# Autodesk Inventor assembly: KND-2610 Main way 01
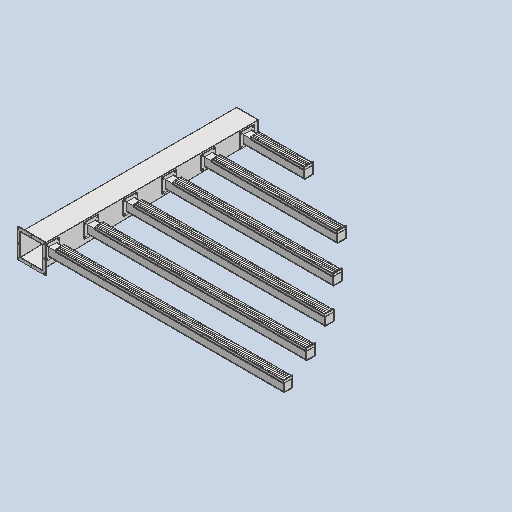
[picture p0: Inventor's stored thumbnail of the model, 512x512]
Saved by Autodesk Inventor 2026.2 (Build 302298000, 298)
## iProperties
Created: 2026-05-12
Part Number: KND-2610 Main way 01
Document SubType Name: Assembly
Designer: admin
Author: admin
## Documents named in this file (19)
- C:\Users\admin\Documents\Inventor\KND-DistribSystem\DRS_D1200\KND-2610 Main way 01.iam
- C:\Users\admin\Documents\Inventor\KND-DistribSystem\DRS_D1200\KND-1425 DrSysB Way FLANGE 01.ipt
- C:\Users\admin\Documents\Inventor\KND-DistribSystem\DRS_D1200\KND-1663 DrSysB way tube 4 01.ipt
- C:\Users\admin\Documents\Inventor\KND-DistribSystem\DRS_D1200\KND-1662 DrSysB way tube 2 01.ipt
- C:\Users\admin\Documents\Inventor\KND-DistribSystem\DRS_D1200\KND-1666 FDS 1000 CUP 1 01.ipt
- C:\Users\admin\Documents\Inventor\KND-DistribSystem\DRS_D1200\KND-1422 DrSysB diameter way up 01.ipt
- C:\Users\admin\Documents\Inventor\KND-DistribSystem\DRS_D1200\KND-1423 DrSysB diameter way down 01.ipt
- C:\Users\admin\Documents\Inventor\KND-DistribSystem\DRS_D1200\KND-1424 DrSysB diam way cup 01.ipt
- C:\Users\admin\Documents\Inventor\KND-DistribSystem\DRS_D1200\KND-1661 DrSysB way tube 1 01.ipt
- C:\Users\admin\Documents\Inventor\KND-DistribSystem\DRS_D1200\KND-5311 DrSysB roof 1 01.ipt
- C:\Users\admin\Documents\Inventor\KND-DistribSystem\DRS_D1200\KND-5321 DrSysB roof 2 01.ipt
- C:\Users\admin\Documents\Inventor\KND-DistribSystem\DRS_D1200\KND-5333 DrSysB roof 3 01.ipt
- C:\Users\admin\Documents\Inventor\KND-DistribSystem\DRS_D1200\KND-1664 DrSysB way tube 44 01.ipt
- C:\Users\admin\Documents\Inventor\KND-DistribSystem\DRS_D1200\KND-5335 DrSysB roof 33 01.ipt
- C:\Users\admin\Documents\Inventor\KND-DistribSystem\DRS_D1200\KND-1667 DrSysB way tube 5 01.ipt
- C:\Users\admin\Documents\Inventor\KND-DistribSystem\DRS_D1200\KND-5337 DrSysB roof 5 01.ipt
- C:\Users\admin\Documents\Inventor\KND-DistribSystem\DRS_D1200\KND-1668 DrSysB way tube 6 01.ipt
- C:\Users\admin\Documents\Inventor\KND-DistribSystem\DRS_D1200\KND-5338 DrSysB roof 6 01.ipt
- C:\Users\admin\Documents\Inventor\KND-DistribSystem\DRS_D1200\KND-1426 DrSysB Main way FLANGE 01.ipt
## Components (28 placed, 20 different names)
1. PRS 1425 DrSysB Way FLANGE_D1200:1 — Mate:34, Mate:40, Mate:41
2. PRS 1662 DrSysB way tube 4_D1200:1 — Mate:55, Mate:56, Mate:57, Mate:70, Flush:12, Mate:80, Mate:81, Flush:17, Mate:89, Flush:24
3. PRS 1662 DrSysB way tube 2_D1200:1 — Mate:52, Mate:53, Mate:54, Mate:67, Mate:68, Flush:11, Mate:78, Mate:79, Flush:16, Mate:88, Flush:22
4. PRS-1666 FDS 1000 CUP 1_D1200:1 — Rigid:17, Mate:15
5. PRS 1422 DrSysB diameter way up_D1200:1 — Flush:10, Flush:9, Mate:11, Rigid:23, Mate:94
6. PRS 1423 DrSysB diameter way down_D1200:1 — Rigid:23, Mate:16, Mate:17, Mate:18, Mate:34, Mate:52, Mate:53, Mate:54, Mate:55, Mate:56, Mate:57, Mate:58, Mate:59, Mate:60, Mate:61, Mate:62, Mate:63, Mate:64, Mate:65, Mate:66, Mate:69, Mate:71, Mate:73, Mate:75, Mate:77, Mate:93, Flush:31
7. PRS 1424 DrSysB diam way cup_D1200:1 — Flush:10, Flush:9, Mate:11
8. PRS 1425 DrSysB Way FLANGE_D1200:2 — Mate:69, Mate:78, Mate:79
9. PRS 1425 DrSysB Way FLANGE_D1200:3 — Mate:71, Mate:80, Mate:81
10. PRS 1661 DrSysB way tube 1_D1200:1 — Rigid:17, Mate:14, Flush:10, Mate:16, Mate:17, Mate:18, Mate:40, Mate:41
11. PRS 5311 DrSysB roof 1_D1200:1 — Mate:14, Flush:10, Mate:15
12. PRS 5321 DrSysB roof 2_D1200:1 — Mate:67, Mate:68, Flush:11, Flush:16, Flush:21
13. PRS 5333 DrSysB roof 3_D1200:1 — Mate:70, Flush:12, Flush:17, Flush:23
14. PRS 1662 DrSysB way tube 44_D1200:1 — Mate:58, Mate:59, Mate:60, Mate:72, Flush:13, Mate:82, Mate:83, Flush:18, Mate:90, Flush:26
15. PRS 5335 DrSysB roof 33_D1200:1 — Mate:72, Flush:13, Flush:18, Flush:25
16. PRS 1425 DrSysB Way FLANGE_D1200:7 — Mate:73, Mate:82, Mate:83
17. KND-1667 DrSysB way tube 5 01:1 — Mate:61, Mate:62, Mate:63, Mate:74, Flush:14, Mate:84, Mate:85, Flush:19, Mate:91, Flush:28
18. KND-5337 DrSysB roof 5 01:1 — Mate:74, Flush:14, Flush:19, Flush:27
19. KND-1425 DrSysB Way FLANGE 01:8 — Mate:75, Mate:84, Mate:85
20. KND-1668 DrSysB way tube 6 01:1 — Mate:64, Mate:65, Mate:66, Mate:76, Flush:15, Mate:86, Mate:87, Flush:20, Mate:92, Flush:30
21. KND-5338 DrSysB roof 6 01:1 — Mate:76, Flush:15, Flush:20, Flush:29
22. KND-1425 DrSysB Way FLANGE 01:9 — Mate:77, Mate:86, Mate:87
23. KND-1666 FDS 1000 CUP 1 01:2 — Mate:88, Flush:21, Flush:22
24. KND-1666 FDS 1000 CUP 1 01:3 — Mate:89, Flush:23, Flush:24
25. KND-1666 FDS 1000 CUP 1 01:4 — Mate:90, Flush:25, Flush:26
26. KND-1666 FDS 1000 CUP 1 01:5 — Mate:91, Flush:27, Flush:28
27. KND-1666 FDS 1000 CUP 1 01:6 — Mate:92, Flush:29, Flush:30
28. KND-1426 DrSysB Main way FLANGE 01:1 — Mate:93, Mate:94, Flush:31
## Relationships (78: Mate 52, Flush 24, WeldJoint 2)
- Flush:10 (1 mm): PRS 1422 DrSysB diameter way up_D1200:1 ↔ PRS 1424 DrSysB diam way cup_D1200:1
- Flush:9 (-1 mm): PRS 1422 DrSysB diameter way up_D1200:1 ↔ PRS 1424 DrSysB diam way cup_D1200:1
- Mate:11: PRS 1422 DrSysB diameter way up_D1200:1 ↔ PRS 1424 DrSysB diam way cup_D1200:1
- Rigid:23 [WeldJoint]: PRS 1422 DrSysB diameter way up_D1200:1 ↔ PRS 1423 DrSysB diameter way down_D1200:1
- Rigid:17 [WeldJoint]: PRS-1666 FDS 1000 CUP 1_D1200:1 ↔ PRS 1661 DrSysB way tube 1_D1200:1
- Mate:14 (10 mm): PRS 1661 DrSysB way tube 1_D1200:1 ↔ PRS 5311 DrSysB roof 1_D1200:1
- Flush:10: PRS 1661 DrSysB way tube 1_D1200:1 ↔ PRS 5311 DrSysB roof 1_D1200:1
- Mate:15: PRS-1666 FDS 1000 CUP 1_D1200:1 ↔ PRS 5311 DrSysB roof 1_D1200:1
- Mate:16: PRS 1423 DrSysB diameter way down_D1200:1 ↔ PRS 1661 DrSysB way tube 1_D1200:1
- Mate:17 (0.25 mm): PRS 1423 DrSysB diameter way down_D1200:1 ↔ PRS 1661 DrSysB way tube 1_D1200:1
- Mate:18 (0.25 mm): PRS 1423 DrSysB diameter way down_D1200:1 ↔ PRS 1661 DrSysB way tube 1_D1200:1
- Mate:34: PRS 1425 DrSysB Way FLANGE_D1200:1 ↔ PRS 1423 DrSysB diameter way down_D1200:1
- Mate:40 (0.1 mm): PRS 1425 DrSysB Way FLANGE_D1200:1 ↔ PRS 1661 DrSysB way tube 1_D1200:1
- Mate:41 (0.1 mm): PRS 1425 DrSysB Way FLANGE_D1200:1 ↔ PRS 1661 DrSysB way tube 1_D1200:1
- Mate:52: PRS 1662 DrSysB way tube 2_D1200:1 ↔ PRS 1423 DrSysB diameter way down_D1200:1
- Mate:53 (0.25 mm): PRS 1662 DrSysB way tube 2_D1200:1 ↔ PRS 1423 DrSysB diameter way down_D1200:1
- Mate:54 (0.25 mm): PRS 1662 DrSysB way tube 2_D1200:1 ↔ PRS 1423 DrSysB diameter way down_D1200:1
- Mate:55: PRS 1662 DrSysB way tube 4_D1200:1 ↔ PRS 1423 DrSysB diameter way down_D1200:1
- Mate:56 (0.25 mm): PRS 1662 DrSysB way tube 4_D1200:1 ↔ PRS 1423 DrSysB diameter way down_D1200:1
- Mate:57 (0.25 mm): PRS 1662 DrSysB way tube 4_D1200:1 ↔ PRS 1423 DrSysB diameter way down_D1200:1
- Mate:58: PRS 1423 DrSysB diameter way down_D1200:1 ↔ PRS 1662 DrSysB way tube 44_D1200:1
- Mate:59 (0.25 mm): PRS 1423 DrSysB diameter way down_D1200:1 ↔ PRS 1662 DrSysB way tube 44_D1200:1
- Mate:60 (0.25 mm): PRS 1423 DrSysB diameter way down_D1200:1 ↔ PRS 1662 DrSysB way tube 44_D1200:1
- Mate:61: PRS 1423 DrSysB diameter way down_D1200:1 ↔ KND-1667 DrSysB way tube 5 01:1
- Mate:62 (0.25 mm): PRS 1423 DrSysB diameter way down_D1200:1 ↔ KND-1667 DrSysB way tube 5 01:1
- Mate:63 (0.25 mm): PRS 1423 DrSysB diameter way down_D1200:1 ↔ KND-1667 DrSysB way tube 5 01:1
- Mate:64: PRS 1423 DrSysB diameter way down_D1200:1 ↔ KND-1668 DrSysB way tube 6 01:1
- Mate:65 (0.25 mm): PRS 1423 DrSysB diameter way down_D1200:1 ↔ KND-1668 DrSysB way tube 6 01:1
- Mate:66 (0.25 mm): PRS 1423 DrSysB diameter way down_D1200:1 ↔ KND-1668 DrSysB way tube 6 01:1
- Mate:67 (10 mm): PRS 1662 DrSysB way tube 2_D1200:1 ↔ PRS 5321 DrSysB roof 2_D1200:1
- Mate:68 (10 mm): PRS 1662 DrSysB way tube 2_D1200:1 ↔ PRS 5321 DrSysB roof 2_D1200:1
- Flush:11: PRS 1662 DrSysB way tube 2_D1200:1 ↔ PRS 5321 DrSysB roof 2_D1200:1
- Mate:69: PRS 1423 DrSysB diameter way down_D1200:1 ↔ PRS 1425 DrSysB Way FLANGE_D1200:2
- Mate:70 (10 mm): PRS 1662 DrSysB way tube 4_D1200:1 ↔ PRS 5333 DrSysB roof 3_D1200:1
- Flush:12: PRS 1662 DrSysB way tube 4_D1200:1 ↔ PRS 5333 DrSysB roof 3_D1200:1
- Mate:71: PRS 1423 DrSysB diameter way down_D1200:1 ↔ PRS 1425 DrSysB Way FLANGE_D1200:3
- Mate:72 (10 mm): PRS 1662 DrSysB way tube 44_D1200:1 ↔ PRS 5335 DrSysB roof 33_D1200:1
- Flush:13: PRS 1662 DrSysB way tube 44_D1200:1 ↔ PRS 5335 DrSysB roof 33_D1200:1
- Mate:73: PRS 1423 DrSysB diameter way down_D1200:1 ↔ PRS 1425 DrSysB Way FLANGE_D1200:7
- Mate:74 (10 mm): KND-1667 DrSysB way tube 5 01:1 ↔ KND-5337 DrSysB roof 5 01:1
- Flush:14: KND-1667 DrSysB way tube 5 01:1 ↔ KND-5337 DrSysB roof 5 01:1
- Mate:75: PRS 1423 DrSysB diameter way down_D1200:1 ↔ KND-1425 DrSysB Way FLANGE 01:8
- Mate:76 (10 mm): KND-1668 DrSysB way tube 6 01:1 ↔ KND-5338 DrSysB roof 6 01:1
- Flush:15: KND-1668 DrSysB way tube 6 01:1 ↔ KND-5338 DrSysB roof 6 01:1
- Mate:77: PRS 1423 DrSysB diameter way down_D1200:1 ↔ KND-1425 DrSysB Way FLANGE 01:9
- Mate:78 (0.1 mm): PRS 1662 DrSysB way tube 2_D1200:1 ↔ PRS 1425 DrSysB Way FLANGE_D1200:2
- Mate:79 (0.1 mm): PRS 1662 DrSysB way tube 2_D1200:1 ↔ PRS 1425 DrSysB Way FLANGE_D1200:2
- Flush:16: PRS 1662 DrSysB way tube 2_D1200:1 ↔ PRS 5321 DrSysB roof 2_D1200:1
- Mate:80 (0.1 mm): PRS 1662 DrSysB way tube 4_D1200:1 ↔ PRS 1425 DrSysB Way FLANGE_D1200:3
- Mate:81 (0.1 mm): PRS 1662 DrSysB way tube 4_D1200:1 ↔ PRS 1425 DrSysB Way FLANGE_D1200:3
- Flush:17: PRS 1662 DrSysB way tube 4_D1200:1 ↔ PRS 5333 DrSysB roof 3_D1200:1
- Mate:82 (0.1 mm): PRS 1662 DrSysB way tube 44_D1200:1 ↔ PRS 1425 DrSysB Way FLANGE_D1200:7
- Mate:83 (0.1 mm): PRS 1662 DrSysB way tube 44_D1200:1 ↔ PRS 1425 DrSysB Way FLANGE_D1200:7
- Flush:18: PRS 1662 DrSysB way tube 44_D1200:1 ↔ PRS 5335 DrSysB roof 33_D1200:1
- Mate:84 (0.1 mm): KND-1667 DrSysB way tube 5 01:1 ↔ KND-1425 DrSysB Way FLANGE 01:8
- Mate:85 (0.1 mm): KND-1667 DrSysB way tube 5 01:1 ↔ KND-1425 DrSysB Way FLANGE 01:8
- Flush:19: KND-1667 DrSysB way tube 5 01:1 ↔ KND-5337 DrSysB roof 5 01:1
- Mate:86 (0.1 mm): KND-1668 DrSysB way tube 6 01:1 ↔ KND-1425 DrSysB Way FLANGE 01:9
- Mate:87 (0.1 mm): KND-1668 DrSysB way tube 6 01:1 ↔ KND-1425 DrSysB Way FLANGE 01:9
- Flush:20: KND-1668 DrSysB way tube 6 01:1 ↔ KND-5338 DrSysB roof 6 01:1
- Mate:88: PRS 1662 DrSysB way tube 2_D1200:1 ↔ KND-1666 FDS 1000 CUP 1 01:2
- Flush:21 (-4.2 mm): PRS 5321 DrSysB roof 2_D1200:1 ↔ KND-1666 FDS 1000 CUP 1 01:2
- Flush:22 (-2.5 mm): PRS 1662 DrSysB way tube 2_D1200:1 ↔ KND-1666 FDS 1000 CUP 1 01:2
- Mate:89: PRS 1662 DrSysB way tube 4_D1200:1 ↔ KND-1666 FDS 1000 CUP 1 01:3
- Flush:23 (-4.2 mm): PRS 5333 DrSysB roof 3_D1200:1 ↔ KND-1666 FDS 1000 CUP 1 01:3
- Flush:24 (-2.5 mm): PRS 1662 DrSysB way tube 4_D1200:1 ↔ KND-1666 FDS 1000 CUP 1 01:3
- Mate:90: PRS 1662 DrSysB way tube 44_D1200:1 ↔ KND-1666 FDS 1000 CUP 1 01:4
- Flush:25 (-4.2 mm): PRS 5335 DrSysB roof 33_D1200:1 ↔ KND-1666 FDS 1000 CUP 1 01:4
- Flush:26 (-2.5 mm): PRS 1662 DrSysB way tube 44_D1200:1 ↔ KND-1666 FDS 1000 CUP 1 01:4
- Mate:91: KND-1667 DrSysB way tube 5 01:1 ↔ KND-1666 FDS 1000 CUP 1 01:5
- Flush:27 (-4.2 mm): KND-5337 DrSysB roof 5 01:1 ↔ KND-1666 FDS 1000 CUP 1 01:5
- Flush:28 (-2.5 mm): KND-1667 DrSysB way tube 5 01:1 ↔ KND-1666 FDS 1000 CUP 1 01:5
- Mate:92: KND-1668 DrSysB way tube 6 01:1 ↔ KND-1666 FDS 1000 CUP 1 01:6
- Flush:29 (-4.2 mm): KND-5338 DrSysB roof 6 01:1 ↔ KND-1666 FDS 1000 CUP 1 01:6
- Flush:30 (-2.5 mm): KND-1668 DrSysB way tube 6 01:1 ↔ KND-1666 FDS 1000 CUP 1 01:6
- Mate:93 (1.1 mm): PRS 1423 DrSysB diameter way down_D1200:1 ↔ KND-1426 DrSysB Main way FLANGE 01:1
- Mate:94 (0.1 mm): PRS 1422 DrSysB diameter way up_D1200:1 ↔ KND-1426 DrSysB Main way FLANGE 01:1
- Flush:31: PRS 1423 DrSysB diameter way down_D1200:1 ↔ KND-1426 DrSysB Main way FLANGE 01:1
